# Autodesk Inventor assembly: Tensioner
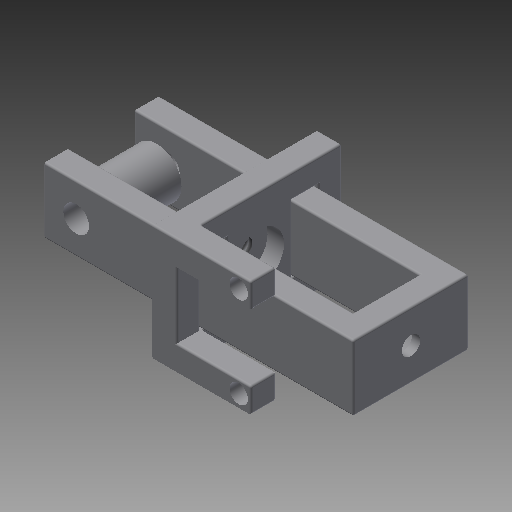
[picture p0: Inventor's stored thumbnail of the model, 512x512]
Saved by Autodesk Inventor 2017 (Build 210142000, 142)
## iProperties
Created: 2017-07-29
Part Number: Tensioner
Document SubType Name: Assembly
Designer: User
Author: User
## Documents named in this file (4)
- C:\Robotics\CAD\2016-17_CAD\DriveTrain\Tensioner.iam
- C:\Robotics\CAD\2016-17_CAD\DriveTrain\TensionerAxleHolder.ipt
- C:\Robotics\CAD\2016-17_CAD\DriveTrain\TensionerPlate.ipt
- C:\Robotics\CAD\2016-17_CAD\Custom COTS\Spacer.188ID.375W.ipt
## Components (3 placed, 3 different names)
1. TensionerAxleHolder:1 — Mate:1, Flush:1, Flush:2
2. TensionerPlate:1 — Mate:1, Flush:1, Flush:2
3. Spacer.188ID.375W:1
## Relationships (3: Flush 2, Mate 1)
- Mate:1: TensionerAxleHolder:1 ↔ TensionerPlate:1
- Flush:1 (4.7625 mm): TensionerAxleHolder:1 ↔ TensionerPlate:1
- Flush:2 (-29.21 mm): TensionerAxleHolder:1 ↔ TensionerPlate:1
